# Autodesk Inventor assembly: X_rail_Assembly_Rev3
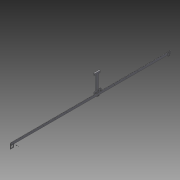
[picture p0: Inventor's stored thumbnail of the model, 180x180]
Saved by Autodesk Inventor 2015 (Build 190159000, 159)
## iProperties
Created: 2017-01-08
Part Number: X_rail_Assembly_Rev3
Document SubType Name: Assembly
Designer: Guy
Author: Guy
## Documents named in this file (10)
- C:\Users\Guy\Documents\Fourth Year\Capstone\git\Capstone-Project\doc\CAD\LowLevel_Rev3\X_rail_Assembly_Rev3.iam
- C:\Users\Guy\Documents\Fourth Year\Capstone\git\Capstone-Project\doc\CAD\LowLevel_Rev3\X_Rai-SquareBar-Rev3.ipt
- C:\Users\Guy\Documents\Fourth Year\Capstone\git\Capstone-Project\doc\CAD\LowLevel_Rev3\XY_Wheel-SquareBar-Rev3.ipt
- C:\Users\Guy\Documents\Fourth Year\Capstone\git\Capstone-Project\doc\CAD\LowLevel_Rev3\Arm_Base-SquareBar-Rev3.ipt
- C:\Users\Guy\Documents\Fourth Year\Capstone\git\Capstone-Project\doc\CAD\LowLevel_Rev3\Arm-SquareBar-Rev3.ipt
- C:\Users\Guy\Documents\Fourth Year\Capstone\git\Capstone-Project\doc\CAD\Nuts and Bolts\3-16in_1 1-4in_Bolt.ipt
- C:\Users\Guy\Documents\Fourth Year\Capstone\git\Capstone-Project\doc\CAD\Nuts and Bolts\3-16in_7-16in_washer(num8).ipt
- C:\Users\Guy\Documents\Fourth Year\Capstone\git\Capstone-Project\doc\CAD\Nuts and Bolts\3-16in_1-16in_nut(num2).ipt
- C:\Users\Guy\Documents\Fourth Year\Capstone\git\Capstone-Project\doc\CAD\Stepper Motor\NEMA 23\NEMA 23 Holder.ipt
- C:\Users\Guy\Documents\Fourth Year\Capstone\git\Capstone-Project\doc\CAD\LowLevel_Rev3\Rail_Pulley_Connector.ipt
## Components (49 placed, 9 different names)
1. X_Rai-SquareBar-Rev3:1 — Tangent:3, Mate:3, Tangent:4, Tangent:5, Mate:86, Mate:87, Mate:88, Mate:89, Mate:90, Mate:105
2. XY_Wheel-SquareBar-Rev3:1 — Tangent:3, Mate:3, Flush:1, Mate:75, Mate:77, Mate:78
3. Arm_Base-SquareBar-Rev3:1 — Mate:10, Mate:15, Mate:16, Mate:17, Mate:18, Mate:19, Mate:20, Mate:21, Mate:22, Mate:23, Mate:24, Mate:25, Mate:26, Mate:27, Mate:44, Mate:45, Mate:47, Mate:65, Mate:66, Mate:67, Mate:76, Mate:79, Mate:82
4. Arm-SquareBar-Rev3:1 — Mate:10, Mate:18, Mate:19, Mate:28, Mate:29, Mate:30, Mate:31
5. XY_Wheel-SquareBar-Rev3:2 — Mate:15, Tangent:4, Flush:2, Mate:17, Mate:68, Mate:69
6. XY_Wheel-SquareBar-Rev3:3 — Mate:16, Tangent:5, Flush:1, Flush:2, Mate:51, Mate:55
7. 3-16in_1 1-4in_Bolt:1 — Mate:20, Mate:21, Mate:40, Mate:41
8. 3-16in_7-16in_washer(num8):1 — Mate:29, Mate:32, Mate:36
9. 3-16in_7-16in_washer(num8):2 — Mate:28, Mate:33, Mate:38
10. 3-16in_7-16in_washer(num8):3 — Mate:30, Mate:35, Mate:40
11. 3-16in_7-16in_washer(num8):4 — Mate:31, Mate:34, Mate:42
12. 3-16in_1 1-4in_Bolt:2 — Mate:24, Mate:26, Mate:36, Mate:37
13. 3-16in_1 1-4in_Bolt:3 — Mate:23, Mate:27, Mate:42, Mate:43
14. 3-16in_1 1-4in_Bolt:4 — Mate:22, Mate:25, Mate:38, Mate:39
15. 3-16in_1-16in_nut(num2):1 — Mate:35, Mate:41
16. 3-16in_1-16in_nut(num2):2 — Mate:34, Mate:43
17. 3-16in_1-16in_nut(num2):3 — Mate:33, Mate:39
18. 3-16in_1-16in_nut(num2):4 — Mate:32, Mate:37
19. 3-16in_1 1-4in_Bolt:5 — Mate:44, Mate:45, Mate:46, Mate:48, Mate:49, Mate:52, Mate:53
20. 3-16in_1 1-4in_Bolt:6 — Mate:60, Mate:61, Mate:62, Mate:63, Mate:64, Mate:65, Mate:66
21. 3-16in_1 1-4in_Bolt:7 — Mate:70, Mate:71, Mate:72, Mate:73, Mate:74, Mate:75, Mate:79, Mate:82
22. 3-16in_1-16in_nut(num2):5 — Mate:46, Mate:47
23. 3-16in_1-16in_nut(num2):6 — Mate:48, Mate:50
24. 3-16in_1-16in_nut(num2):7 — Mate:53, Mate:54
25. 3-16in_7-16in_washer(num8):5 — Mate:49, Mate:50, Mate:55
26. 3-16in_7-16in_washer(num8):6 — Mate:51, Mate:52, Mate:54
27. 3-16in_7-16in_washer(num8):7 — Mate:56, Mate:63, Mate:69
28. 3-16in_7-16in_washer(num8):8 — Mate:57, Mate:61, Mate:68
29. 3-16in_7-16in_washer(num8):9 — Mate:58, Mate:73, Mate:78
30. 3-16in_7-16in_washer(num8):10 — Mate:59, Mate:71, Mate:77
31. 3-16in_1-16in_nut(num2):8 — Mate:56, Mate:64
32. 3-16in_1-16in_nut(num2):9 — Mate:57, Mate:62
33. 3-16in_1-16in_nut(num2):10 — Mate:60, Mate:67
34. 3-16in_1-16in_nut(num2):11 — Mate:58, Mate:74
35. 3-16in_1-16in_nut(num2):12 — Mate:59, Mate:72
36. 3-16in_1-16in_nut(num2):13 — Mate:70, Mate:76
37. NEMA 23 Holder:1 — Mate:86, Mate:87, Mate:88, Mate:106, Mate:107, Mate:113
38. Rail_Pulley_Connector:1 — Mate:89, Mate:90, Mate:92, Mate:94, Mate:104, Mate:105
39. XY_Wheel-SquareBar-Rev3:4 — Mate:93, Mate:101, Mate:102
40. 3-16in_1 1-4in_Bolt:8 — Mate:92, Mate:93, Mate:94, Mate:95, Mate:98, Mate:99, Mate:100, Flush:3
41. 3-16in_1-16in_nut(num2):14 — Mate:97, Mate:103
42. 3-16in_1-16in_nut(num2):15 — Mate:96, Mate:98, Flush:3
43. 3-16in_1-16in_nut(num2):16 — Mate:95, Mate:104
44. 3-16in_7-16in_washer(num8):11 — Mate:97, Mate:99, Mate:102, Mate:103
45. 3-16in_7-16in_washer(num8):12 — Mate:96, Mate:100, Mate:101
46. 3-16in_1 1-4in_Bolt:9 — Mate:106, Mate:107, Mate:109
47. 3-16in_1-16in_nut(num2):17 — Mate:109
48. 3-16in_1 1-4in_Bolt:10 — Mate:111, Mate:113
49. 3-16in_1-16in_nut(num2):18 — Mate:111
## Relationships (98: Mate 92, Tangent 3, Flush 3)
- Tangent:3: X_Rai-SquareBar-Rev3:1 ↔ XY_Wheel-SquareBar-Rev3:1
- Mate:3 (0.075 mm): X_Rai-SquareBar-Rev3:1 ↔ XY_Wheel-SquareBar-Rev3:1
- Mate:10: Arm_Base-SquareBar-Rev3:1 ↔ Arm-SquareBar-Rev3:1
- Mate:15: Arm_Base-SquareBar-Rev3:1 ↔ XY_Wheel-SquareBar-Rev3:2
- Mate:16: Arm_Base-SquareBar-Rev3:1 ↔ XY_Wheel-SquareBar-Rev3:3
- Tangent:4: X_Rai-SquareBar-Rev3:1 ↔ XY_Wheel-SquareBar-Rev3:2
- Tangent:5: X_Rai-SquareBar-Rev3:1 ↔ XY_Wheel-SquareBar-Rev3:3
- Flush:1: XY_Wheel-SquareBar-Rev3:1 ↔ XY_Wheel-SquareBar-Rev3:3
- Flush:2: XY_Wheel-SquareBar-Rev3:2 ↔ XY_Wheel-SquareBar-Rev3:3
- Mate:17 (7 mm): Arm_Base-SquareBar-Rev3:1 ↔ XY_Wheel-SquareBar-Rev3:2
- Mate:18: Arm_Base-SquareBar-Rev3:1 ↔ Arm-SquareBar-Rev3:1
- Mate:19: Arm_Base-SquareBar-Rev3:1 ↔ Arm-SquareBar-Rev3:1
- Mate:20: Arm_Base-SquareBar-Rev3:1 ↔ 3-16in_1 1-4in_Bolt:1
- Mate:21: Arm_Base-SquareBar-Rev3:1 ↔ 3-16in_1 1-4in_Bolt:1
- Mate:22: Arm_Base-SquareBar-Rev3:1 ↔ 3-16in_1 1-4in_Bolt:4
- Mate:23: Arm_Base-SquareBar-Rev3:1 ↔ 3-16in_1 1-4in_Bolt:3
- Mate:24: Arm_Base-SquareBar-Rev3:1 ↔ 3-16in_1 1-4in_Bolt:2
- Mate:25: Arm_Base-SquareBar-Rev3:1 ↔ 3-16in_1 1-4in_Bolt:4
- Mate:26: Arm_Base-SquareBar-Rev3:1 ↔ 3-16in_1 1-4in_Bolt:2
- Mate:27: Arm_Base-SquareBar-Rev3:1 ↔ 3-16in_1 1-4in_Bolt:3
- Mate:28: Arm-SquareBar-Rev3:1 ↔ 3-16in_7-16in_washer(num8):2
- Mate:29: Arm-SquareBar-Rev3:1 ↔ 3-16in_7-16in_washer(num8):1
- Mate:30: Arm-SquareBar-Rev3:1 ↔ 3-16in_7-16in_washer(num8):3
- Mate:31: Arm-SquareBar-Rev3:1 ↔ 3-16in_7-16in_washer(num8):4
- Mate:32: 3-16in_7-16in_washer(num8):1 ↔ 3-16in_1-16in_nut(num2):4
- Mate:33: 3-16in_7-16in_washer(num8):2 ↔ 3-16in_1-16in_nut(num2):3
- Mate:34: 3-16in_7-16in_washer(num8):4 ↔ 3-16in_1-16in_nut(num2):2
- Mate:35: 3-16in_7-16in_washer(num8):3 ↔ 3-16in_1-16in_nut(num2):1
- Mate:36: 3-16in_7-16in_washer(num8):1 ↔ 3-16in_1 1-4in_Bolt:2
- Mate:37: 3-16in_1 1-4in_Bolt:2 ↔ 3-16in_1-16in_nut(num2):4
- Mate:38: 3-16in_7-16in_washer(num8):2 ↔ 3-16in_1 1-4in_Bolt:4
- Mate:39: 3-16in_1 1-4in_Bolt:4 ↔ 3-16in_1-16in_nut(num2):3
- Mate:40: 3-16in_1 1-4in_Bolt:1 ↔ 3-16in_7-16in_washer(num8):3
- Mate:41: 3-16in_1 1-4in_Bolt:1 ↔ 3-16in_1-16in_nut(num2):1
- Mate:42: 3-16in_7-16in_washer(num8):4 ↔ 3-16in_1 1-4in_Bolt:3
- Mate:43: 3-16in_1 1-4in_Bolt:3 ↔ 3-16in_1-16in_nut(num2):2
- Mate:44: Arm_Base-SquareBar-Rev3:1 ↔ 3-16in_1 1-4in_Bolt:5
- Mate:45: Arm_Base-SquareBar-Rev3:1 ↔ 3-16in_1 1-4in_Bolt:5
- Mate:46: 3-16in_1 1-4in_Bolt:5 ↔ 3-16in_1-16in_nut(num2):5
- Mate:47: Arm_Base-SquareBar-Rev3:1 ↔ 3-16in_1-16in_nut(num2):5
- Mate:48: 3-16in_1 1-4in_Bolt:5 ↔ 3-16in_1-16in_nut(num2):6
- Mate:49: 3-16in_1 1-4in_Bolt:5 ↔ 3-16in_7-16in_washer(num8):5
- Mate:50: 3-16in_1-16in_nut(num2):6 ↔ 3-16in_7-16in_washer(num8):5
- Mate:51: XY_Wheel-SquareBar-Rev3:3 ↔ 3-16in_7-16in_washer(num8):6
- Mate:52: 3-16in_1 1-4in_Bolt:5 ↔ 3-16in_7-16in_washer(num8):6
- Mate:53: 3-16in_1 1-4in_Bolt:5 ↔ 3-16in_1-16in_nut(num2):7
- Mate:54: 3-16in_1-16in_nut(num2):7 ↔ 3-16in_7-16in_washer(num8):6
- Mate:55: XY_Wheel-SquareBar-Rev3:3 ↔ 3-16in_7-16in_washer(num8):5
- Mate:56: 3-16in_7-16in_washer(num8):7 ↔ 3-16in_1-16in_nut(num2):8
- Mate:57: 3-16in_7-16in_washer(num8):8 ↔ 3-16in_1-16in_nut(num2):9
- Mate:58: 3-16in_7-16in_washer(num8):9 ↔ 3-16in_1-16in_nut(num2):11
- Mate:59: 3-16in_7-16in_washer(num8):10 ↔ 3-16in_1-16in_nut(num2):12
- Mate:60: 3-16in_1 1-4in_Bolt:6 ↔ 3-16in_1-16in_nut(num2):10
- Mate:61: 3-16in_1 1-4in_Bolt:6 ↔ 3-16in_7-16in_washer(num8):8
- Mate:62: 3-16in_1 1-4in_Bolt:6 ↔ 3-16in_1-16in_nut(num2):9
- Mate:63: 3-16in_1 1-4in_Bolt:6 ↔ 3-16in_7-16in_washer(num8):7
- Mate:64: 3-16in_1 1-4in_Bolt:6 ↔ 3-16in_1-16in_nut(num2):8
- Mate:65: Arm_Base-SquareBar-Rev3:1 ↔ 3-16in_1 1-4in_Bolt:6
- Mate:66: Arm_Base-SquareBar-Rev3:1 ↔ 3-16in_1 1-4in_Bolt:6
- Mate:67: Arm_Base-SquareBar-Rev3:1 ↔ 3-16in_1-16in_nut(num2):10
- Mate:68: XY_Wheel-SquareBar-Rev3:2 ↔ 3-16in_7-16in_washer(num8):8
- Mate:69: XY_Wheel-SquareBar-Rev3:2 ↔ 3-16in_7-16in_washer(num8):7
- Mate:70: 3-16in_1 1-4in_Bolt:7 ↔ 3-16in_1-16in_nut(num2):13
- Mate:71: 3-16in_1 1-4in_Bolt:7 ↔ 3-16in_7-16in_washer(num8):10
- Mate:72: 3-16in_1 1-4in_Bolt:7 ↔ 3-16in_1-16in_nut(num2):12
- Mate:73: 3-16in_1 1-4in_Bolt:7 ↔ 3-16in_7-16in_washer(num8):9
- Mate:74: 3-16in_1 1-4in_Bolt:7 ↔ 3-16in_1-16in_nut(num2):11
- Mate:75: XY_Wheel-SquareBar-Rev3:1 ↔ 3-16in_1 1-4in_Bolt:7
- Mate:76: Arm_Base-SquareBar-Rev3:1 ↔ 3-16in_1-16in_nut(num2):13
- Mate:77: XY_Wheel-SquareBar-Rev3:1 ↔ 3-16in_7-16in_washer(num8):10
- Mate:78: XY_Wheel-SquareBar-Rev3:1 ↔ 3-16in_7-16in_washer(num8):9
- Mate:79: Arm_Base-SquareBar-Rev3:1 ↔ 3-16in_1 1-4in_Bolt:7
- Mate:82: Arm_Base-SquareBar-Rev3:1 ↔ 3-16in_1 1-4in_Bolt:7
- Mate:86: X_Rai-SquareBar-Rev3:1 ↔ NEMA 23 Holder:1
- Mate:87: X_Rai-SquareBar-Rev3:1 ↔ NEMA 23 Holder:1
- Mate:88: X_Rai-SquareBar-Rev3:1 ↔ NEMA 23 Holder:1
- Mate:89: X_Rai-SquareBar-Rev3:1 ↔ Rail_Pulley_Connector:1
- Mate:90: X_Rai-SquareBar-Rev3:1 ↔ Rail_Pulley_Connector:1
- Mate:92: Rail_Pulley_Connector:1 ↔ 3-16in_1 1-4in_Bolt:8
- Mate:93: XY_Wheel-SquareBar-Rev3:4 ↔ 3-16in_1 1-4in_Bolt:8
- Mate:94: Rail_Pulley_Connector:1 ↔ 3-16in_1 1-4in_Bolt:8
- Mate:95: 3-16in_1 1-4in_Bolt:8 ↔ 3-16in_1-16in_nut(num2):16
- Mate:96: 3-16in_1-16in_nut(num2):15 ↔ 3-16in_7-16in_washer(num8):12
- Mate:97: 3-16in_1-16in_nut(num2):14 ↔ 3-16in_7-16in_washer(num8):11
- Mate:98: 3-16in_1 1-4in_Bolt:8 ↔ 3-16in_1-16in_nut(num2):15
- Mate:99: 3-16in_1 1-4in_Bolt:8 ↔ 3-16in_7-16in_washer(num8):11
- Mate:100: 3-16in_1 1-4in_Bolt:8 ↔ 3-16in_7-16in_washer(num8):12
- Mate:101: XY_Wheel-SquareBar-Rev3:4 ↔ 3-16in_7-16in_washer(num8):12
- Mate:102: XY_Wheel-SquareBar-Rev3:4 ↔ 3-16in_7-16in_washer(num8):11
- Mate:103: 3-16in_1-16in_nut(num2):14 ↔ 3-16in_7-16in_washer(num8):11
- Mate:104: Rail_Pulley_Connector:1 ↔ 3-16in_1-16in_nut(num2):16
- Flush:3 (5 mm): 3-16in_1 1-4in_Bolt:8 ↔ 3-16in_1-16in_nut(num2):15
- Mate:105: X_Rai-SquareBar-Rev3:1 ↔ Rail_Pulley_Connector:1
- Mate:106: NEMA 23 Holder:1 ↔ 3-16in_1 1-4in_Bolt:9
- Mate:107: NEMA 23 Holder:1 ↔ 3-16in_1 1-4in_Bolt:9
- Mate:109: 3-16in_1 1-4in_Bolt:9 ↔ 3-16in_1-16in_nut(num2):17
- Mate:111: 3-16in_1 1-4in_Bolt:10 ↔ 3-16in_1-16in_nut(num2):18
- Mate:113: NEMA 23 Holder:1 ↔ 3-16in_1 1-4in_Bolt:10
